# Autodesk Inventor assembly: RF_Rover_Motor2_liegend
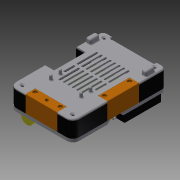
[picture p0: Inventor's stored thumbnail of the model, 180x180]
Saved by Autodesk Inventor 2015 (Build 190159000, 159)
## iProperties
Created: 2015-03-02
Part Number: RF_Rover_Motor2_liegend
Document SubType Name: Assembly
Designer: TowerSebi
Author: TowerSebi
## Documents named in this file (12)
- C:\Users\krumms\Documents\Inventor\Laborarbeit\RF_Rover_Motor2_liegend.iam
- C:\Users\krumms\Documents\Inventor\Laborarbeit\Bodenplatte_Motor2_liegend.ipt
- C:\Users\krumms\Documents\Inventor\Laborarbeit\Deckel_Motor2_liegend.ipt
- C:\Users\krumms\Documents\Inventor\Laborarbeit\Peripherie_Motor2_liegend.ipt
- C:\Users\krumms\Documents\Inventor\Laborarbeit\Zwischenebene_Motor2_liegend.ipt
- C:\Users\krumms\Documents\Inventor\Laborarbeit\Motor_gerade.ipt
- C:\Users\krumms\Documents\Inventor\Laborarbeit\Batteriehalter_6AA.ipt
- C:\Users\krumms\Documents\Inventor\Laborarbeit\stiftleiste.ipt
- C:\Users\krumms\Documents\Inventor\Laborarbeit\Peripherie2_Motor2_liegend.ipt
- C:\Users\krumms\Documents\Inventor\Laborarbeit\SMD_Platine.ipt
- C:\Users\krumms\Documents\Inventor\Laborarbeit\Testplatine.ipt
- C:\Users\krumms\Documents\Inventor\Laborarbeit\Deckel2_Motor2_liegend.ipt
## Components (16 placed, 11 different names)
1. Bodenplatte_Motor2_liegend:1 — Passend:1, Passend:2, Passend:4, Passend:5, Passend:6, Passend:7, Passend:8, Passend:9, Passend:10, Passend:11, Passend:12, Passend:13, Passend:19, Passend:20, Passend:21, Passend:22, Passend:23, Passend:24, Passend:25, Passend:26, Passend:27, Passend:34, Passend:35, Passend:36, Passend:37, Passend:38, Passend:39, Passend:40, Passend:41, Passend:42, Passend:43, Fluchtend:4, Passend:50
2. Deckel_Motor2_liegend:1 — Passend:14, Passend:45, Passend:46, Passend:47, Passend:48
3. Peripherie_Motor2_liegend:1 — Passend:5, Passend:6, Passend:13
4. Zwischenebene_Motor2_liegend:1 — Passend:1, Passend:2, Passend:4, Passend:14, Passend:28, Fluchtend:1, Passend:29, Passend:30, Fluchtend:2, Passend:32, Fluchtend:3, Passend:33, Passend:44, Passend:45, Passend:46, Passend:47, Passend:48, Fluchtend:5, Passend:49
5. Peripherie_Motor2_liegend:2 — Passend:9, Passend:10, Passend:11
6. Peripherie_Motor2_liegend:3 — Passend:7, Passend:8, Passend:12
7. Motor_gerade:1 — Passend:20, Passend:23, Passend:24
8. Motor_gerade:2 — Passend:19, Passend:21, Passend:22
9. Batteriehalter_6AA:1 — Passend:25, Passend:26, Passend:27
10. stiftleiste:1 — Passend:30, Fluchtend:2, Passend:44
11. stiftleiste:2 — Passend:28, Fluchtend:1, Passend:29
12. stiftleiste:3 — Passend:32, Fluchtend:3, Passend:33
13. Peripherie2_Motor2_liegend:1 — Passend:34, Passend:35, Passend:36, Passend:50
14. SMD_Platine:1 — Passend:41, Passend:42, Passend:43
15. Testplatine:1 — Passend:37, Passend:38, Passend:39, Passend:40
16. Deckel2_Motor2_liegend:1 — Fluchtend:4, Fluchtend:5, Passend:49
## Relationships (49: Mate 44, Flush 5)
- Passend:1 [Mate]: Bodenplatte_Motor2_liegend:1 ↔ Zwischenebene_Motor2_liegend:1
- Passend:2 [Mate]: Bodenplatte_Motor2_liegend:1 ↔ Zwischenebene_Motor2_liegend:1
- Passend:4 [Mate]: Bodenplatte_Motor2_liegend:1 ↔ Zwischenebene_Motor2_liegend:1
- Passend:5 [Mate]: Bodenplatte_Motor2_liegend:1 ↔ Peripherie_Motor2_liegend:1
- Passend:6 [Mate]: Bodenplatte_Motor2_liegend:1 ↔ Peripherie_Motor2_liegend:1
- Passend:7 [Mate]: Bodenplatte_Motor2_liegend:1 ↔ Peripherie_Motor2_liegend:3
- Passend:8 [Mate]: Bodenplatte_Motor2_liegend:1 ↔ Peripherie_Motor2_liegend:3
- Passend:9 [Mate]: Bodenplatte_Motor2_liegend:1 ↔ Peripherie_Motor2_liegend:2
- Passend:10 [Mate]: Bodenplatte_Motor2_liegend:1 ↔ Peripherie_Motor2_liegend:2
- Passend:11 [Mate]: Bodenplatte_Motor2_liegend:1 ↔ Peripherie_Motor2_liegend:2
- Passend:12 [Mate]: Bodenplatte_Motor2_liegend:1 ↔ Peripherie_Motor2_liegend:3
- Passend:13 [Mate]: Bodenplatte_Motor2_liegend:1 ↔ Peripherie_Motor2_liegend:1
- Passend:14 [Mate]: Deckel_Motor2_liegend:1 ↔ Zwischenebene_Motor2_liegend:1
- Passend:19 [Mate]: Bodenplatte_Motor2_liegend:1 ↔ Motor_gerade:2
- Passend:20 [Mate]: Bodenplatte_Motor2_liegend:1 ↔ Motor_gerade:1
- Passend:21 [Mate]: Bodenplatte_Motor2_liegend:1 ↔ Motor_gerade:2
- Passend:22 [Mate]: Bodenplatte_Motor2_liegend:1 ↔ Motor_gerade:2
- Passend:23 [Mate]: Bodenplatte_Motor2_liegend:1 ↔ Motor_gerade:1
- Passend:24 [Mate]: Bodenplatte_Motor2_liegend:1 ↔ Motor_gerade:1
- Passend:25 [Mate]: Bodenplatte_Motor2_liegend:1 ↔ Batteriehalter_6AA:1
- Passend:26 [Mate]: Bodenplatte_Motor2_liegend:1 ↔ Batteriehalter_6AA:1
- Passend:27 [Mate]: Bodenplatte_Motor2_liegend:1 ↔ Batteriehalter_6AA:1
- Passend:28 [Mate]: Zwischenebene_Motor2_liegend:1 ↔ stiftleiste:2
- Fluchtend:1 [Flush]: Zwischenebene_Motor2_liegend:1 ↔ stiftleiste:2
- Passend:29 [Mate]: Zwischenebene_Motor2_liegend:1 ↔ stiftleiste:2
- Passend:30 [Mate]: Zwischenebene_Motor2_liegend:1 ↔ stiftleiste:1
- Fluchtend:2 [Flush]: Zwischenebene_Motor2_liegend:1 ↔ stiftleiste:1
- Passend:32 [Mate]: Zwischenebene_Motor2_liegend:1 ↔ stiftleiste:3
- Fluchtend:3 [Flush]: Zwischenebene_Motor2_liegend:1 ↔ stiftleiste:3
- Passend:33 [Mate]: Zwischenebene_Motor2_liegend:1 ↔ stiftleiste:3
- Passend:34 [Mate]: Bodenplatte_Motor2_liegend:1 ↔ Peripherie2_Motor2_liegend:1
- Passend:35 [Mate]: Bodenplatte_Motor2_liegend:1 ↔ Peripherie2_Motor2_liegend:1
- Passend:36 [Mate]: Bodenplatte_Motor2_liegend:1 ↔ Peripherie2_Motor2_liegend:1
- Passend:37 [Mate]: Bodenplatte_Motor2_liegend:1 ↔ Testplatine:1
- Passend:38 [Mate] (10 mm): Bodenplatte_Motor2_liegend:1 ↔ Testplatine:1
- Passend:39 [Mate]: Bodenplatte_Motor2_liegend:1 ↔ Testplatine:1
- Passend:40 [Mate]: Bodenplatte_Motor2_liegend:1 ↔ Testplatine:1
- Passend:41 [Mate]: Bodenplatte_Motor2_liegend:1 ↔ SMD_Platine:1
- Passend:42 [Mate]: Bodenplatte_Motor2_liegend:1 ↔ SMD_Platine:1
- Passend:43 [Mate] (10 mm): Bodenplatte_Motor2_liegend:1 ↔ SMD_Platine:1
- Passend:44 [Mate]: Zwischenebene_Motor2_liegend:1 ↔ stiftleiste:1
- Passend:45 [Mate]: Deckel_Motor2_liegend:1 ↔ Zwischenebene_Motor2_liegend:1
- Passend:46 [Mate]: Deckel_Motor2_liegend:1 ↔ Zwischenebene_Motor2_liegend:1
- Passend:47 [Mate]: Deckel_Motor2_liegend:1 ↔ Zwischenebene_Motor2_liegend:1
- Passend:48 [Mate]: Deckel_Motor2_liegend:1 ↔ Zwischenebene_Motor2_liegend:1
- Fluchtend:4 [Flush]: Bodenplatte_Motor2_liegend:1 ↔ Deckel2_Motor2_liegend:1
- Fluchtend:5 [Flush]: Zwischenebene_Motor2_liegend:1 ↔ Deckel2_Motor2_liegend:1
- Passend:49 [Mate]: Zwischenebene_Motor2_liegend:1 ↔ Deckel2_Motor2_liegend:1
- Passend:50 [Mate]: Bodenplatte_Motor2_liegend:1 ↔ Peripherie2_Motor2_liegend:1
